# Autodesk Inventor assembly: Weapon (Weapon-Side Pulley)
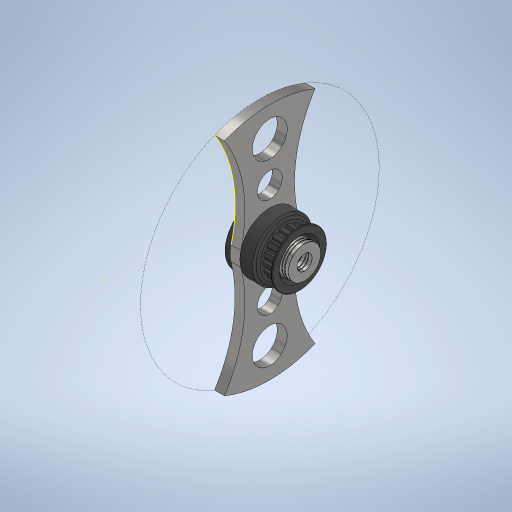
[picture p0: Inventor's stored thumbnail of the model, 512x512]
Saved by Autodesk Inventor 2023.1 (Build 271208000, 208)
## iProperties
Created: 2022-05-08
Part Number: Weapon (Weapon-Side Pulley)
Document SubType Name: Assembly
Designer: NCai2
Mass: 280.359 g
Surface Area: 311.324 cm^2
Volume: 49.83 cm^3
Density: 5.62632 g/cm^3
Author: NCai2
## Documents named in this file (6)
- E:\Documents\Inventor\0.3rd Lawette - V3.4\Vertical Weapon Assembly (Type A)\Weapon (Weapon-Side Pulley).iam
- E:\Documents\Inventor\0.3rd Lawette - V3.4\Vertical Weapon Assembly (Type A)\Thrust Ball Bearing.ipt
- E:\Documents\Inventor\0.3rd Lawette - V3.4\Vertical Weapon Assembly (Type A)\5905K132_Needle-Roller Bearing.ipt
- E:\Documents\Inventor\0.3rd Lawette - V3.4\Vertical Weapon Assembly (Type A)\Spacer 3-8x .125.ipt
- E:\Documents\Inventor\0.3rd Lawette - V3.4\Vertical Weapon Assembly (Type A)\Blade (Bar 2).ipt
- E:\Documents\Inventor\0.3rd Lawette - V3.4\Vertical Weapon Assembly (Type A)\XL Pulley 18T .25in Wd.ipt
## Components (7 placed, 5 different names)
1. 5905K132_Needle-Roller Bearing:3 — Mate:12, Mate:14, Mate:15, Mate:18, Mate:31
2. 5905K132_Needle-Roller Bearing:4 — Mate:9, Mate:13, Mate:15, Mate:17, Mate:31
3. Thrust Ball Bearing:3 — Mate:9, Mate:16, Mate:17
4. Thrust Ball Bearing:4 — Mate:12, Mate:14, Mate:16, Mate:21, Mate:28
5. Blade (Bar 2):1 — Mate:13, Mate:19, Mate:20, Mate:29, Mate:30
6. Spacer 3-8x .125:1 — Mate:18, Mate:19, Mate:20, Mate:21
7. XL Pulley 18T .25in Wd:1 — Mate:28, Mate:29, Mate:30
## Relationships (15: Mate 15)
- Mate:9: 5905K132_Needle-Roller Bearing:4 ↔ Thrust Ball Bearing:3
- Mate:12: 5905K132_Needle-Roller Bearing:3 ↔ Thrust Ball Bearing:4
- Mate:13: 5905K132_Needle-Roller Bearing:4 ↔ Blade (Bar 2):1
- Mate:14: 5905K132_Needle-Roller Bearing:3 ↔ Thrust Ball Bearing:4
- Mate:15: 5905K132_Needle-Roller Bearing:3 ↔ 5905K132_Needle-Roller Bearing:4
- Mate:16 (-38.1 mm): Thrust Ball Bearing:3 ↔ Thrust Ball Bearing:4
- Mate:17: 5905K132_Needle-Roller Bearing:4 ↔ Thrust Ball Bearing:3
- Mate:18: 5905K132_Needle-Roller Bearing:3 ↔ Spacer 3-8x .125:1
- Mate:19: Blade (Bar 2):1 ↔ Spacer 3-8x .125:1
- Mate:20: Blade (Bar 2):1 ↔ Spacer 3-8x .125:1
- Mate:21: Thrust Ball Bearing:4 ↔ Spacer 3-8x .125:1
- Mate:28 (-34.925 mm): Thrust Ball Bearing:4 ↔ XL Pulley 18T .25in Wd:1
- Mate:29: Blade (Bar 2):1 ↔ XL Pulley 18T .25in Wd:1
- Mate:30: Blade (Bar 2):1 ↔ XL Pulley 18T .25in Wd:1
- Mate:31: 5905K132_Needle-Roller Bearing:3 ↔ 5905K132_Needle-Roller Bearing:4
